# Autodesk Inventor assembly: Sneak100_Zeta
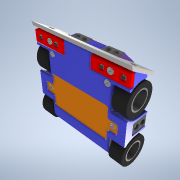
[picture p0: Inventor's stored thumbnail of the model, 180x180]
Saved by Autodesk Inventor 2021 (Build 250183000, 183)
## iProperties
Created: 2021-05-13
Part Number: Sneak100_Zeta
Document SubType Name: Assembly
Designer: ermoz
Author: ermoz
## iProperties of the stored document proxima_kicadSOLID_5.ipt
Created: 2021-08-02
Part Number: proxima_kicadSOLID_5
Material: Generic
Document SubType Name: Modeling
Designer: ermoz
Density: 1 g/cm^3
Appearance: Default
Author: ermoz
## iProperties of the stored document proxima_kicadLED_0805_2012Metric.iam
Created: 2021-08-02
Part Number: proxima_kicadLED_0805_2012Metric
Document SubType Name: Assembly
Designer: ermoz
Author: ermoz
## iProperties of the stored document proxima_case.ipt
Created: 2021-08-02
Part Number: proxima_case
Material: Generic
Document SubType Name: Modeling
Designer: ermoz
Density: 1 g/cm^3
Appearance: Default
Author: ermoz
## iProperties of the stored document proxima_kicadSOLID_3.ipt
Created: 2021-08-02
Part Number: proxima_kicadSOLID_3
Material: Generic
Document SubType Name: Modeling
Designer: ermoz
Density: 1 g/cm^3
Appearance: Default
Author: ermoz
## iProperties of the stored document proxima_kicadCP_EIA-3216-10_Kemet-I.iam
Created: 2021-08-02
Part Number: proxima_kicadCP_EIA-3216-10_Kemet-I
Document SubType Name: Assembly
Designer: ermoz
Author: ermoz
## iProperties of the stored document proxima_kicadSOLID_2.ipt
Created: 2021-08-02
Part Number: proxima_kicadSOLID_2
Material: Generic
Document SubType Name: Modeling
Designer: ermoz
Density: 1 g/cm^3
Appearance: Default
Author: ermoz
## iProperties of the stored document proxima_kicadCOMPOUND.ipt
Created: 2021-08-02
Part Number: proxima_kicadCOMPOUND
Material: Generic
Document SubType Name: Modeling
Designer: ermoz
Density: 1 g/cm^3
Appearance: Default
Author: ermoz
## iProperties of the stored document proxima_sensor_model.iam
Created: 2021-08-02
Part Number: proxima_sensor_model
Document SubType Name: Assembly
Designer: ermoz
Sending System: Autodesk Inventor 2021
Preprocessor: ST-DEVELOPER v18.1
Title: D:\Moje Wyczyny\My_Poor_Projects\Proxima_sensor\proxima-sensor\version_1.xx\proxima_sensor_case\proxima_sensor_model.stp
Author: ermoz
## iProperties of the stored document proxima_kicadVishay_MOLD-3Pin.iam
Created: 2021-08-02
Part Number: proxima_kicadVishay_MOLD-3Pin
Document SubType Name: Assembly
Designer: ermoz
Author: ermoz
## iProperties of the stored document proxima_kicadSOLID_4.ipt
Created: 2021-08-02
Part Number: proxima_kicadSOLID_4
Material: Generic
Document SubType Name: Modeling
Designer: ermoz
Density: 1 g/cm^3
Appearance: Default
Author: ermoz
## iProperties of the stored document proxima_kicadproxima_sensor_board.iam
Created: 2021-08-02
Part Number: proxima_kicadproxima_sensor_board
Document SubType Name: Assembly
Designer: ermoz
Author: ermoz
## iProperties of the stored document proxima_kicadR_0805_2012Metric.iam
Created: 2021-08-02
Part Number: proxima_kicadR_0805_2012Metric
Document SubType Name: Assembly
Designer: ermoz
Author: ermoz
## iProperties of the stored document proxima_kicadSOLID_1.ipt
Created: 2021-08-02
Part Number: proxima_kicadSOLID_1
Material: Generic
Document SubType Name: Modeling
Designer: ermoz
Density: 1 g/cm^3
Appearance: Default
Author: ermoz
## iProperties of the stored document proxima_kicadC_0805_2012Metric.iam
Created: 2021-08-02
Part Number: proxima_kicadC_0805_2012Metric
Document SubType Name: Assembly
Designer: ermoz
Author: ermoz
## iProperties of the stored document proxima_kicadSOLID_7.ipt
Created: 2021-08-02
Part Number: proxima_kicadSOLID_7
Material: Generic
Document SubType Name: Modeling
Designer: ermoz
Density: 1 g/cm^3
Appearance: Default
Author: ermoz
## iProperties of the stored document proxima_kicadSOIC-8_3.9x4.9mm_P1.27mm.iam
Created: 2021-08-02
Part Number: proxima_kicadSOIC-8_3.9x4.9mm_P1.27mm
Document SubType Name: Assembly
Designer: ermoz
Author: ermoz
## iProperties of the stored document proxima_kicadLED_D5.0mm_IRGrey.iam
Created: 2021-08-02
Part Number: proxima_kicadLED_D5.0mm_IRGrey
Document SubType Name: Assembly
Designer: ermoz
Author: ermoz
## iProperties of the stored document proxima_kicadSOLID_6.ipt
Created: 2021-08-02
Part Number: proxima_kicadSOLID_6
Material: Generic
Document SubType Name: Modeling
Designer: ermoz
Density: 1 g/cm^3
Appearance: Default
Author: ermoz
## Documents named in this file (36)
- D:\Moje Wyczyny\My_Poor_Projects\Sneak100_MiniSumo\minisumo-sneak100\mechanics\Sneak100_Zeta.iam
- D:\Moje Wyczyny\My_Poor_Projects\Sneak100_MiniSumo\minisumo-sneak100\mechanics\PreMadeParts\Pololu_MotorEncoderModule.iam
- D:\Moje Wyczyny\My_Poor_Projects\Sneak100_MiniSumo\minisumo-sneak100\mechanics\ElectricElements\LiPO_2S_58x32x10.ipt
- D:\Moje Wyczyny\My_Poor_Projects\Sneak100_MiniSumo\minisumo-sneak100\mechanics\PreMadeParts\Solarbotics_RW2i.ipt
- D:\Moje Wyczyny\My_Poor_Projects\Sneak100_MiniSumo\minisumo-sneak100\mechanics\MechanicalElements\HullBottom.ipt
- D:\Moje Wyczyny\My_Poor_Projects\Sneak100_MiniSumo\minisumo-sneak100\mechanics\MechanicalElements\BatteryPlate.ipt
- D:\Moje Wyczyny\My_Poor_Projects\Sneak100_MiniSumo\minisumo-sneak100\mechanics\ElectricElements\QTR1A.iam
- D:\Moje Wyczyny\My_Poor_Projects\Sneak100_MiniSumo\minisumo-sneak100\mechanics\PreMadeParts\M3_Short_Bolt.ipt
- D:\Moje Wyczyny\My_Poor_Projects\Sneak100_MiniSumo\minisumo-sneak100\mechanics\ModyfiedParts\HM_Knife_cut.ipt
- D:\Moje Wyczyny\My_Poor_Projects\Sneak100_MiniSumo\minisumo-sneak100\mechanics\PreMadeParts\3M_Nut.ipt
- D:\Moje Wyczyny\My_Poor_Projects\Sneak100_MiniSumo\minisumo-sneak100\mechanics\MechanicalElements\HullMid.ipt
- D:\Moje Wyczyny\My_Poor_Projects\Sneak100_MiniSumo\minisumo-sneak100\mechanics\MirroredParts\HullMid_MIR.ipt
- D:\Moje Wyczyny\My_Poor_Projects\Sneak100_MiniSumo\minisumo-sneak100\mechanics\MechanicalElements\HullTop.ipt
- D:\Moje Wyczyny\My_Poor_Projects\Sneak100_MiniSumo\minisumo-sneak100\mechanics\ElectricElements\MainModule.iam
- D:\Moje Wyczyny\My_Poor_Projects\Sneak100_MiniSumo\minisumo-sneak100\mechanics\PreMadeParts\M3_Long_Bolt.ipt
- D:\Moje Wyczyny\My_Poor_Projects\Sneak100_MiniSumo\minisumo-sneak100\mechanics\ElectricElements\HC-05_module.iam
- **D:\Moje Wyczyny\My_Poor_Projects\Sneak100_MiniSumo\minisumo-sneak100\mechanics\Sneak100_Zeta.iam*LocalDocs*xAaaaagdaAaaaaaaaAaaaq2kyBd*proxima_sensor_model.iam
- D:\Moje Wyczyny\My_Poor_Projects\Sneak100_MiniSumo\minisumo-sneak100\mechanics\MechanicalElements\LineSensorPlate.ipt
- D:\Moje Wyczyny\My_Poor_Projects\Sneak100_MiniSumo\minisumo-sneak100\mechanics\ElectricElements\proxima_sensor_model.stp
- **D:\Moje Wyczyny\My_Poor_Projects\Sneak100_MiniSumo\minisumo-sneak100\mechanics\Sneak100_Zeta.iam*LocalDocs*xAaaaahbaAaaaaaaaAaaaaig44h*proxima_kicadSOLID_5.ipt
- **D:\Moje Wyczyny\My_Poor_Projects\Sneak100_MiniSumo\minisumo-sneak100\mechanics\Sneak100_Zeta.iam*LocalDocs*xAaaaa5daAaaaaaaaAaaaamfbYd*proxima_kicadLED_0805_2012Metric.iam
- **D:\Moje Wyczyny\My_Poor_Projects\Sneak100_MiniSumo\minisumo-sneak100\mechanics\Sneak100_Zeta.iam*LocalDocs*xAaaaa2caAaaaaaaaAaaaqec31a*proxima_case.ipt
- **D:\Moje Wyczyny\My_Poor_Projects\Sneak100_MiniSumo\minisumo-sneak100\mechanics\Sneak100_Zeta.iam*LocalDocs*xAaaaa1caAaaaaaaaAaaaqsvxMh*proxima_kicadSOLID_3.ipt
- **D:\Moje Wyczyny\My_Poor_Projects\Sneak100_MiniSumo\minisumo-sneak100\mechanics\Sneak100_Zeta.iam*LocalDocs*xAaaaa5aaAaaaaaaaAaaaay5l4e*proxima_kicadCP_EIA-3216-10_Kemet-I.iam
- **D:\Moje Wyczyny\My_Poor_Projects\Sneak100_MiniSumo\minisumo-sneak100\mechanics\Sneak100_Zeta.iam*LocalDocs*xAaaaazbaAaaaaaaaAaaaaptw0e*proxima_kicadSOLID_1.ipt
- **D:\Moje Wyczyny\My_Poor_Projects\Sneak100_MiniSumo\minisumo-sneak100\mechanics\Sneak100_Zeta.iam*LocalDocs*xAaaaafaaAaaaaaaaAaaaqw4nTa*proxima_kicadSOLID_2.ipt
- **D:\Moje Wyczyny\My_Poor_Projects\Sneak100_MiniSumo\minisumo-sneak100\mechanics\Sneak100_Zeta.iam*LocalDocs*xAaaaabaaAaaaaaaaAaaaqc4uUd*proxima_kicadCOMPOUND.ipt
- **D:\Moje Wyczyny\My_Poor_Projects\Sneak100_MiniSumo\minisumo-sneak100\mechanics\Sneak100_Zeta.iam*LocalDocs*xAaaaajdaAaaaaaaaAaaaqs2cHf*proxima_kicadproxima_sensor_board.iam
- **D:\Moje Wyczyny\My_Poor_Projects\Sneak100_MiniSumo\minisumo-sneak100\mechanics\Sneak100_Zeta.iam*LocalDocs*xAaaaauaaAaaaaaaaAaaaakq2Ta*proxima_kicadVishay_MOLD-3Pin.iam
- **D:\Moje Wyczyny\My_Poor_Projects\Sneak100_MiniSumo\minisumo-sneak100\mechanics\Sneak100_Zeta.iam*LocalDocs*xAaaaakdaAaaaaaaaAaaaa1kjFd*proxima_kicadSOLID_4.ipt
- **D:\Moje Wyczyny\My_Poor_Projects\Sneak100_MiniSumo\minisumo-sneak100\mechanics\Sneak100_Zeta.iam*LocalDocs*xAaaaqabaAaaaaaaaAaaaqqsoVc*proxima_kicadSOIC-8_3.9x4.9mm_P1.27mm.iam
- **D:\Moje Wyczyny\My_Poor_Projects\Sneak100_MiniSumo\minisumo-sneak100\mechanics\Sneak100_Zeta.iam*LocalDocs*xAaaaancaAaaaaaaaAaaaq3wnJb*proxima_kicadR_0805_2012Metric.iam
- **D:\Moje Wyczyny\My_Poor_Projects\Sneak100_MiniSumo\minisumo-sneak100\mechanics\Sneak100_Zeta.iam*LocalDocs*xAaaaqoaaAaaaaaaaAaaaa51tDd*proxima_kicadLED_D5.0mm_IRGrey.iam
- **D:\Moje Wyczyny\My_Poor_Projects\Sneak100_MiniSumo\minisumo-sneak100\mechanics\Sneak100_Zeta.iam*LocalDocs*xAaaaaycaAaaaaaaaAaaaanxhSa*proxima_kicadC_0805_2012Metric.iam
- **D:\Moje Wyczyny\My_Poor_Projects\Sneak100_MiniSumo\minisumo-sneak100\mechanics\Sneak100_Zeta.iam*LocalDocs*xAaaaqddaAaaaaaaaAaaaaktrQc*proxima_kicadSOLID_7.ipt
- **D:\Moje Wyczyny\My_Poor_Projects\Sneak100_MiniSumo\minisumo-sneak100\mechanics\Sneak100_Zeta.iam*LocalDocs*xAaaaqtcaAaaaaaaaAaaaanvkXh*proxima_kicadSOLID_6.ipt
## Components (51 placed, 17 different names)
1. Pololu_MotorEncoderModule:1 [sub-assembly] — Mate:89, Mate:90, Flush:42, Mate:96
2. Pololu_MotorEncoderModule:2 [sub-assembly] — Angle:2, Mate:9, Mate:16, Mate:95, Flush:45
3. Pololu_MotorEncoderModule:3 [sub-assembly] — Mate:8, Mate:91, Mate:92, Flush:43
4. Pololu_MotorEncoderModule:4 [sub-assembly] — Mate:10, Mate:93, Mate:94, Flush:44
5. LiPO_2S_58x32x10:1 — Mate:17, Mate:18
6. Solarbotics_RW2i:1 — Mate:3, Tangent:1, Flush:8, Symmetry:2, Mate:96
7. Solarbotics_RW2i:2 — Tangent:2, Mate:9, Flush:8, Flush:11, Tangent:3
8. Solarbotics_RW2i:3 — Mate:3, Mate:8, Flush:7, Symmetry:2, Flush:22
9. Solarbotics_RW2i:4 — Mate:10, Flush:7
10. HullBottom:1 — Flush:11, Mate:16, Mate:17, Mate:18, Flush:29, Flush:31, Mate:47, Mate:48, Flush:33, Mate:52, Mate:56, Mate:74, Flush:39, Mate:80, Mate:83, Mate:84, Mate:87, Mate:89, Mate:90, Flush:42, Mate:91, Mate:92, Flush:43, Mate:93, Mate:94, Flush:44, Mate:95, Flush:45, Mate:97, Mate:98, Mate:102, Flush:52, Mate:104, Mate:105, Mate:106, Flush:53, Flush:54, Mate:111, Mate:112, Mate:113, Mate:114, Mate:115, Flush:55, Mate:117, Mate:118, Mate:119, Mate:121, Mate:122, Mate:123, Mate:124, Flush:58, Flush:59, Mate:134, Mate:137, Mate:141, Mate:142
11. LineSensorPlate:1 — Flush:59, Mate:128, Mate:129, Flush:60, Mate:132, Mate:133, Flush:62, Mate:134, Mate:136, Flush:64, Mate:137
12. LineSensorPlate:2 — Flush:58, Mate:126, Mate:127, Flush:60, Mate:130, Mate:131, Flush:62, Mate:135, Flush:63
13. QTR1A:1 [sub-assembly] — Mate:129, Mate:133
14. QTR1A:2 [sub-assembly] — Mate:128, Mate:132
15. QTR1A:3 [sub-assembly] — Mate:126, Mate:131
16. QTR1A:4 [sub-assembly] — Mate:127, Mate:130
17. M3_Short_Bolt:5 — Flush:23, Mate:31
18. M3_Short_Bolt:6 — Flush:24, Mate:85, Mate:143
19. HM_Knife_cut:1 — Flush:22, Flush:23, Mate:31, Flush:24, Mate:80, Mate:88, Mate:143
20. HullMid:1 — Mate:45, Mate:51, Mate:55, Flush:38, Mate:72, Mate:74, Flush:55
21. HullMid_MIR:1 — Flush:29, Mate:43, Mate:59, Flush:38, Mate:73, Flush:46
22. BatteryPlate:1 — Mate:117, Mate:118, Flush:56, Mate:122, Flush:57
23. HullTop:1 — Flush:31, Mate:61, Flush:39, Mate:115
24. MainModule:1 [sub-assembly] — Mate:43, Mate:45, Mate:72, Mate:73, Flush:46, Mate:99, Mate:100, Mate:101
25. M3_Long_Bolt:1 — Mate:47, Flush:32, Flush:33, Mate:49, Mate:60
26. M3_Long_Bolt:2 — Mate:48, Flush:32, Mate:50, Mate:63
27. M3_Long_Bolt:3 — Mate:52, Mate:54, Mate:62, Mate:97
28. M3_Long_Bolt:4 — Mate:56, Mate:58, Mate:64, Mate:98
29. 3M_Nut:7 — Mate:49, Flush:34, Mate:51
30. 3M_Nut:8 — Mate:50, Flush:34
31. 3M_Nut:9 — Mate:54, Mate:55
32. 3M_Nut:10 — Mate:58, Mate:59
33. 3M_Nut:11 — Mate:60, Flush:35, Mate:61, Flush:37
34. 3M_Nut:12 — Mate:63, Flush:37
35. 3M_Nut:13 — Flush:35, Mate:62, Flush:36
36. 3M_Nut:14 — Flush:36, Mate:64
37. 3M_Nut:15 — Mate:85, Mate:87
38. 3M_Nut:16 — Mate:83, Mate:84
39. HC-05_module:1 [sub-assembly] — Mate:99, Mate:100, Mate:101
40. proxima_sensor_model:1 [sub-assembly] — Flush:53, Mate:111, Mate:112
41. proxima_sensor_model:2 [sub-assembly] — Flush:50, Mate:102, Flush:52, Mate:104
42. proxima_sensor_model:3 [sub-assembly] — Flush:50, Mate:105, Mate:106
43. proxima_sensor_model:4 [sub-assembly] — Flush:54, Mate:113, Mate:114
44. M3_Short_Bolt:7 — Mate:119, Flush:56, Mate:120
45. 3M_Nut:17 — Mate:120, Mate:121
46. 3M_Nut:18 — Mate:123, Mate:124, Mate:125
47. M3_Short_Bolt:8 — Mate:125, Flush:57
48. M3_Short_Bolt:9 — Mate:135, Flush:63, Mate:138
49. M3_Short_Bolt:10 — Mate:136, Flush:64, Mate:139
50. 3M_Nut:19 — Mate:138, Mate:142
51. 3M_Nut:20 — Mate:139, Mate:141
## Relationships (122: Mate 83, Flush 34, Tangent 3, Angle 1, Symmetry 1)
- Mate:3 (-98 mm): Solarbotics_RW2i:1 ↔ Solarbotics_RW2i:3
- Tangent:1: Solarbotics_RW2i:1
- Angle:2 (0 deg): Pololu_MotorEncoderModule:2
- Tangent:2: Solarbotics_RW2i:2
- Mate:8: Pololu_MotorEncoderModule:3 ↔ Solarbotics_RW2i:3
- Mate:9: Pololu_MotorEncoderModule:2 ↔ Solarbotics_RW2i:2
- Mate:10: Pololu_MotorEncoderModule:4 ↔ Solarbotics_RW2i:4
- Flush:7: Solarbotics_RW2i:3 ↔ Solarbotics_RW2i:4
- Flush:8: Solarbotics_RW2i:1 ↔ Solarbotics_RW2i:2
- Symmetry:2: Solarbotics_RW2i:1 ↔ Solarbotics_RW2i:3
- Flush:11: Solarbotics_RW2i:2 ↔ HullBottom:1
- Mate:16: Pololu_MotorEncoderModule:2 ↔ HullBottom:1
- Mate:17: LiPO_2S_58x32x10:1 ↔ HullBottom:1
- Mate:18 (1 mm): LiPO_2S_58x32x10:1 ↔ HullBottom:1
- Flush:22 (-1 mm): Solarbotics_RW2i:3 ↔ HM_Knife_cut:1
- Flush:23: M3_Short_Bolt:5 ↔ HM_Knife_cut:1
- Mate:31: M3_Short_Bolt:5 ↔ HM_Knife_cut:1
- Flush:24: M3_Short_Bolt:6 ↔ HM_Knife_cut:1
- Flush:29: HullBottom:1 ↔ HullMid_MIR:1
- Mate:43: HullMid_MIR:1 ↔ MainModule:1
- Mate:45: HullMid:1 ↔ MainModule:1
- Flush:31: HullBottom:1 ↔ HullTop:1
- Mate:47: HullBottom:1 ↔ M3_Long_Bolt:1
- Mate:48: HullBottom:1 ↔ M3_Long_Bolt:2
- Flush:32: M3_Long_Bolt:1 ↔ M3_Long_Bolt:2
- Flush:33: HullBottom:1 ↔ M3_Long_Bolt:1
- Mate:49: M3_Long_Bolt:1 ↔ 3M_Nut:7
- Mate:50: M3_Long_Bolt:2 ↔ 3M_Nut:8
- Flush:34: 3M_Nut:7 ↔ 3M_Nut:8
- Mate:51: HullMid:1 ↔ 3M_Nut:7
- Mate:52: HullBottom:1 ↔ M3_Long_Bolt:3
- Mate:54: M3_Long_Bolt:3 ↔ 3M_Nut:9
- Mate:55: HullMid:1 ↔ 3M_Nut:9
- Mate:56: HullBottom:1 ↔ M3_Long_Bolt:4
- Mate:58: M3_Long_Bolt:4 ↔ 3M_Nut:10
- Mate:59: HullMid_MIR:1 ↔ 3M_Nut:10
- Mate:60: M3_Long_Bolt:1 ↔ 3M_Nut:11
- Flush:35: 3M_Nut:11 ↔ 3M_Nut:13
- Mate:61: HullTop:1 ↔ 3M_Nut:11
- Mate:62: M3_Long_Bolt:3 ↔ 3M_Nut:13
- Flush:36: 3M_Nut:13 ↔ 3M_Nut:14
- Mate:63: M3_Long_Bolt:2 ↔ 3M_Nut:12
- Flush:37: 3M_Nut:11 ↔ 3M_Nut:12
- Mate:64: M3_Long_Bolt:4 ↔ 3M_Nut:14
- Flush:38: HullMid:1 ↔ HullMid_MIR:1
- Mate:72: HullMid:1 ↔ MainModule:1
- Mate:73: HullMid_MIR:1 ↔ MainModule:1
- Mate:74: HullBottom:1 ↔ HullMid:1
- Flush:39: HullBottom:1 ↔ HullTop:1
- Mate:80: HullBottom:1 ↔ HM_Knife_cut:1
- Tangent:3: Solarbotics_RW2i:2
- Mate:83: HullBottom:1 ↔ 3M_Nut:16
- Mate:84: HullBottom:1 ↔ 3M_Nut:16
- Mate:85: M3_Short_Bolt:6 ↔ 3M_Nut:15
- Mate:87: HullBottom:1 ↔ 3M_Nut:15
- Mate:88: HM_Knife_cut:1
- Mate:89: Pololu_MotorEncoderModule:1 ↔ HullBottom:1
- Mate:90 (0.1 mm): Pololu_MotorEncoderModule:1 ↔ HullBottom:1
- Flush:42: Pololu_MotorEncoderModule:1 ↔ HullBottom:1
- Mate:91: Pololu_MotorEncoderModule:3 ↔ HullBottom:1
- Mate:92 (0.1 mm): Pololu_MotorEncoderModule:3 ↔ HullBottom:1
- Flush:43: Pololu_MotorEncoderModule:3 ↔ HullBottom:1
- Mate:93: Pololu_MotorEncoderModule:4 ↔ HullBottom:1
- Mate:94 (0.1 mm): Pololu_MotorEncoderModule:4 ↔ HullBottom:1
- Flush:44: Pololu_MotorEncoderModule:4 ↔ HullBottom:1
- Mate:95 (0.1 mm): Pololu_MotorEncoderModule:2 ↔ HullBottom:1
- Flush:45: Pololu_MotorEncoderModule:2 ↔ HullBottom:1
- Mate:96: Pololu_MotorEncoderModule:1 ↔ Solarbotics_RW2i:1
- Mate:97: HullBottom:1 ↔ M3_Long_Bolt:3
- Mate:98: HullBottom:1 ↔ M3_Long_Bolt:4
- Flush:46: HullMid_MIR:1 ↔ MainModule:1
- Mate:99: MainModule:1 ↔ HC-05_module:1
- Mate:100: MainModule:1 ↔ HC-05_module:1
- Mate:101: MainModule:1 ↔ HC-05_module:1
- Flush:50: proxima_sensor_model:2 ↔ proxima_sensor_model:3
- Mate:102 (0.25 mm): HullBottom:1 ↔ proxima_sensor_model:2
- Flush:52: HullBottom:1 ↔ proxima_sensor_model:2
- Mate:104 (0.25 mm): HullBottom:1 ↔ proxima_sensor_model:2
- Mate:105 (0.25 mm): HullBottom:1 ↔ proxima_sensor_model:3
- Mate:106 (0.25 mm): HullBottom:1 ↔ proxima_sensor_model:3
- Flush:53: HullBottom:1 ↔ proxima_sensor_model:1
- Flush:54: HullBottom:1 ↔ proxima_sensor_model:4
- Mate:111: HullBottom:1 ↔ proxima_sensor_model:1
- Mate:112 (0.25 mm): HullBottom:1 ↔ proxima_sensor_model:1
- Mate:113: HullBottom:1 ↔ proxima_sensor_model:4
- Mate:114 (0.25 mm): HullBottom:1 ↔ proxima_sensor_model:4
- Mate:115: HullBottom:1 ↔ HullTop:1
- Flush:55: HullBottom:1 ↔ HullMid:1
- Mate:117 (0.25 mm): HullBottom:1 ↔ BatteryPlate:1
- Mate:118 (0.5 mm): HullBottom:1 ↔ BatteryPlate:1
- Mate:119: HullBottom:1 ↔ M3_Short_Bolt:7
- Flush:56: BatteryPlate:1 ↔ M3_Short_Bolt:7
- Mate:120: M3_Short_Bolt:7 ↔ 3M_Nut:17
- Mate:121: HullBottom:1 ↔ 3M_Nut:17
- Mate:122: HullBottom:1 ↔ BatteryPlate:1
- Mate:123: HullBottom:1 ↔ 3M_Nut:18
- Mate:124: HullBottom:1 ↔ 3M_Nut:18
- Mate:125: 3M_Nut:18 ↔ M3_Short_Bolt:8
- Flush:57: BatteryPlate:1 ↔ M3_Short_Bolt:8
- Flush:58: HullBottom:1 ↔ LineSensorPlate:2
- Flush:59: HullBottom:1 ↔ LineSensorPlate:1
- Mate:126: LineSensorPlate:2 ↔ QTR1A:3
- Mate:127: LineSensorPlate:2 ↔ QTR1A:4
- Mate:128: LineSensorPlate:1 ↔ QTR1A:2
- Mate:129: LineSensorPlate:1 ↔ QTR1A:1
- Flush:60: LineSensorPlate:1 ↔ LineSensorPlate:2
- Mate:130: LineSensorPlate:2 ↔ QTR1A:4
- Mate:131: LineSensorPlate:2 ↔ QTR1A:3
- Mate:132: LineSensorPlate:1 ↔ QTR1A:2
- Mate:133: LineSensorPlate:1 ↔ QTR1A:1
- Flush:62: LineSensorPlate:1 ↔ LineSensorPlate:2
- Mate:134: HullBottom:1 ↔ LineSensorPlate:1
- Mate:135: LineSensorPlate:2 ↔ M3_Short_Bolt:9
- Mate:136: LineSensorPlate:1 ↔ M3_Short_Bolt:10
- Flush:63: LineSensorPlate:2 ↔ M3_Short_Bolt:9
- Flush:64: LineSensorPlate:1 ↔ M3_Short_Bolt:10
- Mate:137: HullBottom:1 ↔ LineSensorPlate:1
- Mate:138: M3_Short_Bolt:9 ↔ 3M_Nut:19
- Mate:139: M3_Short_Bolt:10 ↔ 3M_Nut:20
- Mate:141: HullBottom:1 ↔ 3M_Nut:20
- Mate:142: HullBottom:1 ↔ 3M_Nut:19
- Mate:143: M3_Short_Bolt:6 ↔ HM_Knife_cut:1
